# Autodesk Inventor assembly: BaseDrive Frame
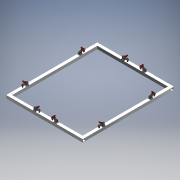
[picture p0: Inventor's stored thumbnail of the model, 180x180]
Saved by Autodesk Inventor 2018 (Build 220112000, 112)
## iProperties
Created: 2018-01-13
Part Number: BaseDrive Frame
Document SubType Name: Assembly
Designer: s-4000369
Author: s-4000369
## Documents named in this file (5)
- C:\Users\S-2512711\Desktop\Drivebase 2018 Files Final Kinda\Drivebase 2018 Files Final Kinda\Drivebase 2018 Files 2\Drivebase 2018 Files 2\BaseDrive\BaseDrive\BaseDrive Frame.iam
- C:\Users\S-2512711\Desktop\Drivebase 2018 Files Final Kinda\Drivebase 2018 Files Final Kinda\Drivebase 2018 Files 2\Drivebase 2018 Files 2\BaseDrive\BaseDrive\1by1by31.ipt
- C:\Users\S-2512711\Desktop\Drivebase 2018 Files Final Kinda\Drivebase 2018 Files Final Kinda\Drivebase 2018 Files 2\Drivebase 2018 Files 2\BaseDrive\BaseDrive\1by1by26.ipt
- C:\Users\S-2512711\Desktop\Drivebase 2018 Files Final Kinda\Drivebase 2018 Files Final Kinda\Drivebase 2018 Files 2\Drivebase 2018 Files 2\BaseDrive\BaseDrive\1by1by6.ipt
- C:\Users\S-2512711\Desktop\Drivebase 2018 Files Final Kinda\Drivebase 2018 Files Final Kinda\Drivebase 2018 Files 2\Drivebase 2018 Files 2\AIS2018\305-U.iam
## Components (12 placed, 4 different names)
1. 1by1by31:1 — Mate:1, Mate:2, Mate:3, Mate:7, Mate:8, Mate:9, Mate:25, Mate:26, Rotation:7, Mate:27, Mate:28, Rotation:8
2. 1by1by26:1 — Mate:1, Mate:2, Mate:3, Mate:13, Mate:14, Rotation:1, Mate:15, Mate:16, Rotation:2
3. 1by1by26:2 — Mate:7, Mate:8, Mate:9, Mate:10, Mate:11, Mate:12, Mate:21, Mate:22, Rotation:5, Mate:23, Mate:24, Rotation:6
4. 1by1by6:1 — Mate:10, Mate:11, Mate:12, Mate:17, Mate:18, Rotation:3, Mate:19, Mate:20, Rotation:4
5. 305-U:1 [sub-assembly] — Mate:13, Mate:14, Rotation:1
6. 305-U:2 [sub-assembly] — Mate:21, Mate:22, Rotation:5
7. 305-U:3 [sub-assembly] — Mate:27, Mate:28, Rotation:8
8. 305-U:4 [sub-assembly] — Mate:17, Mate:18, Rotation:3
9. 305-U:5 [sub-assembly] — Mate:15, Mate:16, Rotation:2
10. 305-U:6 [sub-assembly] — Mate:23, Mate:24, Rotation:6
11. 305-U:7 [sub-assembly] — Mate:25, Mate:26, Rotation:7
12. 305-U:8 [sub-assembly] — Mate:19, Mate:20, Rotation:4
## Relationships (33: Mate 25, RelateRotation 8)
- Mate:1: 1by1by31:1 ↔ 1by1by26:1
- Mate:2: 1by1by31:1 ↔ 1by1by26:1
- Mate:3: 1by1by31:1 ↔ 1by1by26:1
- Mate:7: 1by1by31:1 ↔ 1by1by26:2
- Mate:8: 1by1by31:1 ↔ 1by1by26:2
- Mate:9: 1by1by31:1 ↔ 1by1by26:2
- Mate:10: 1by1by26:2 ↔ 1by1by6:1
- Mate:11: 1by1by26:2 ↔ 1by1by6:1
- Mate:12: 1by1by26:2 ↔ 1by1by6:1
- Mate:13: 1by1by26:1 ↔ 305-U:1
- Mate:14: 1by1by26:1 ↔ 305-U:1
- Rotation:1 [RelateRotation] (1.001 ul): 1by1by26:1 ↔ 305-U:1
- Mate:15: 1by1by26:1 ↔ 305-U:5
- Mate:16: 1by1by26:1 ↔ 305-U:5
- Rotation:2 [RelateRotation] (1.001 ul): 1by1by26:1 ↔ 305-U:5
- Mate:17: 1by1by6:1 ↔ 305-U:4
- Mate:18: 1by1by6:1 ↔ 305-U:4
- Rotation:3 [RelateRotation] (1.001 ul): 1by1by6:1 ↔ 305-U:4
- Mate:19: 1by1by6:1 ↔ 305-U:8
- Mate:20: 1by1by6:1 ↔ 305-U:8
- Rotation:4 [RelateRotation] (0.999 ul): 1by1by6:1 ↔ 305-U:8
- Mate:21: 1by1by26:2 ↔ 305-U:2
- Mate:22: 1by1by26:2 ↔ 305-U:2
- Rotation:5 [RelateRotation] (1.001 ul): 1by1by26:2 ↔ 305-U:2
- Mate:23: 1by1by26:2 ↔ 305-U:6
- Mate:24: 1by1by26:2 ↔ 305-U:6
- Rotation:6 [RelateRotation] (1 ul): 1by1by26:2 ↔ 305-U:6
- Mate:25: 1by1by31:1 ↔ 305-U:7
- Mate:26: 1by1by31:1 ↔ 305-U:7
- Rotation:7 [RelateRotation] (1.001 ul): 1by1by31:1 ↔ 305-U:7
- Mate:27: 1by1by31:1 ↔ 305-U:3
- Mate:28: 1by1by31:1 ↔ 305-U:3
- Rotation:8 [RelateRotation] (1.001 ul): 1by1by31:1 ↔ 305-U:3
